# Autodesk Inventor assembly: v5马达+螺丝
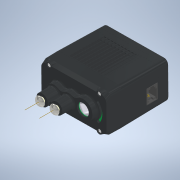
[picture p0: Inventor's stored thumbnail of the model, 180x180]
Saved by Autodesk Inventor 2020 (Build 240168000, 168)
## iProperties
Created: 2019-05-29
Part Number: v5马达+螺丝
Document SubType Name: Assembly
Designer: aresp
Author: aresp
## Documents named in this file (3)
- D:\vault\ncrCadLib\V5主控系统\v5马达+螺丝.iam
- D:\vault\ncrCadLib\V5主控系统\V5_Smart_Motor_276-4840.iam
- D:\vault\ncrCadLib\螺丝螺帽\Screw 8-32 x 0.500'' 三号.ipt
## Components (3 placed, 2 different names)
1. V5_Smart_Motor_276-4840:1 [sub-assembly] — 配合:1, 配合:2, 配合:3
2. Screw 8-32 x 0.500'' 三号:1 — 配合:1, 表面齐平:1, 配合:3
3. Screw 8-32 x 0.500'' 三号:2 — 配合:2, 表面齐平:1
## Relationships (4: Mate 3, Flush 1)
- 配合:1 [Mate]: V5_Smart_Motor_276-4840:1 ↔ Screw 8-32 x 0.500'' 三号:1
- 配合:2 [Mate]: V5_Smart_Motor_276-4840:1 ↔ Screw 8-32 x 0.500'' 三号:2
- 表面齐平:1 [Flush]: Screw 8-32 x 0.500'' 三号:1 ↔ Screw 8-32 x 0.500'' 三号:2
- 配合:3 [Mate] (1.5748 mm): V5_Smart_Motor_276-4840:1 ↔ Screw 8-32 x 0.500'' 三号:1
